# Autodesk Inventor assembly: Ensamblaje_Carcaza_sup_ch
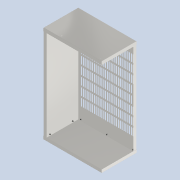
[picture p0: Inventor's stored thumbnail of the model, 180x180]
Saved by Autodesk Inventor 2021 (Build 250183000, 183)
## iProperties
Created: 2021-05-16
Part Number: Ensamblaje_Carcaza_sup_ch
Document SubType Name: Assembly
Designer: Admin
Mass: 2946.62 g
Surface Area: 11445.5 cm^2
Volume: 374.317 cm^3
Density: 7.872 g/cm^3
Author: Admin
## Documents named in this file (7)
- E:\Documentos\Documentos\Michael_Rodriguez\Universidad_Nacional\Doceaba matricula\PAI\Proyecto PAI\Proyecto_PAI_2021\01 CAD\Ensamblaje_Carcaza_sup_ch.iam
- E:\Documentos\Documentos\Michael_Rodriguez\Universidad_Nacional\Doceaba matricula\PAI\Proyecto PAI\Proyecto_PAI_2021\01 CAD\Tapa_superior_sup_ch.ipt
- E:\Documentos\Documentos\Michael_Rodriguez\Universidad_Nacional\Doceaba matricula\PAI\Proyecto PAI\Proyecto_PAI_2021\01 CAD\Tapa_superior_izq_ch.ipt
- E:\Documentos\Documentos\Michael_Rodriguez\Universidad_Nacional\Doceaba matricula\PAI\Proyecto PAI\Proyecto_PAI_2021\01 CAD\Tapa_superior_der_ch.ipt
- E:\Documentos\Documentos\Michael_Rodriguez\Universidad_Nacional\Doceaba matricula\PAI\Proyecto PAI\Proyecto_PAI_2021\01 CAD\ISO 7380-1 - M5 x 8.ipt
- E:\Documentos\Documentos\Michael_Rodriguez\Universidad_Nacional\Doceaba matricula\PAI\Proyecto PAI\Proyecto_PAI_2021\01 CAD\BS 4320 - M5 (Forma A).ipt
- E:\Documentos\Documentos\Michael_Rodriguez\Universidad_Nacional\Doceaba matricula\PAI\Proyecto PAI\Proyecto_PAI_2021\01 CAD\BS 4183 - M5(1).ipt
## Components (33 placed, 6 different names)
1. Tapa_superior_sup_ch:1 — Coincidencia:1, Coincidencia:2, Coincidencia:3, Coincidencia:4, Coincidencia:5, Coincidencia:6, De rotación:21, De rotación:22, De rotación:23, De rotación:24, De rotación:25, De rotación:26, De rotación:27, De rotación:28, De rotación:29, De rotación:30
2. Tapa_superior_izq_ch:1 — Coincidencia:4, Coincidencia:5, Coincidencia:6, De rotación:1, De rotación:2, De rotación:3, De rotación:13, De rotación:14
3. Tapa_superior_der_ch:1 — Coincidencia:1, Coincidencia:2, Coincidencia:3, De rotación:4, De rotación:5, De rotación:6, De rotación:15, De rotación:16
4. ISO 7380-1 M5 x 8:1 — De rotación:8
5. ISO 7380-1 M5 x 8:2 — De rotación:9
6. ISO 7380-1 M5 x 8:3 — De rotación:12
7. ISO 7380-1 M5 x 8:4 — De rotación:7
8. ISO 7380-1 M5 x 8:5 — De rotación:10
9. ISO 7380-1 M5 x 8:6 — De rotación:11
10. ISO 7380-1 M5 x 8:7 — De rotación:17
11. ISO 7380-1 M5 x 8:8 — De rotación:19
12. ISO 7380-1 M5 x 8:9 — De rotación:18
13. ISO 7380-1 M5 x 8:10 — De rotación:20
14. BS 4320 Forma AB M5 (Forma A):1 — De rotación:6, De rotación:12
15. BS 4320 Forma AB M5 (Forma A):2 — De rotación:5, De rotación:11
16. BS 4320 Forma AB M5 (Forma A):3 — De rotación:4, De rotación:10
17. BS 4320 Forma AB M5 (Forma A):4 — De rotación:3, De rotación:9
18. BS 4320 Forma AB M5 (Forma A):5 — De rotación:2, De rotación:8
19. BS 4320 Forma AB M5 (Forma A):6 — De rotación:1, De rotación:7
20. BS 4320 Forma AB M5 (Forma A):7 — De rotación:13, De rotación:17
21. BS 4320 Forma AB M5 (Forma A):8 — De rotación:14, De rotación:18
22. BS 4320 Forma AB M5 (Forma A):9 — De rotación:15, De rotación:20
23. BS 4320 Forma AB M5 (Forma A):10 — De rotación:16, De rotación:19
24. BS 4183 - Métrico M5:1 — De rotación:21
25. BS 4183 - Métrico M5:2 — De rotación:23
26. BS 4183 - Métrico M5:3 — De rotación:26
27. BS 4183 - Métrico M5:4 — De rotación:22
28. BS 4183 - Métrico M5:5 — De rotación:24
29. BS 4183 - Métrico M5:6 — De rotación:25
30. BS 4183 - Métrico M5:7 — De rotación:27
31. BS 4183 - Métrico M5:8 — De rotación:29
32. BS 4183 - Métrico M5:9 — De rotación:28
33. BS 4183 - Métrico M5:10 — De rotación:30
## Relationships (36: RevoluteJoint 30, Mate 6)
- Coincidencia:1 [Mate]: Tapa_superior_sup_ch:1 ↔ Tapa_superior_der_ch:1
- Coincidencia:2 [Mate]: Tapa_superior_sup_ch:1 ↔ Tapa_superior_der_ch:1
- Coincidencia:3 [Mate]: Tapa_superior_sup_ch:1 ↔ Tapa_superior_der_ch:1
- Coincidencia:4 [Mate]: Tapa_superior_sup_ch:1 ↔ Tapa_superior_izq_ch:1
- Coincidencia:5 [Mate]: Tapa_superior_sup_ch:1 ↔ Tapa_superior_izq_ch:1
- Coincidencia:6 [Mate]: Tapa_superior_sup_ch:1 ↔ Tapa_superior_izq_ch:1
- De rotación:1 [RevoluteJoint]: Tapa_superior_izq_ch:1 ↔ BS 4320 Forma AB M5 (Forma A):6
- De rotación:2 [RevoluteJoint]: Tapa_superior_izq_ch:1 ↔ BS 4320 Forma AB M5 (Forma A):5
- De rotación:3 [RevoluteJoint]: Tapa_superior_izq_ch:1 ↔ BS 4320 Forma AB M5 (Forma A):4
- De rotación:4 [RevoluteJoint]: Tapa_superior_der_ch:1 ↔ BS 4320 Forma AB M5 (Forma A):3
- De rotación:5 [RevoluteJoint]: Tapa_superior_der_ch:1 ↔ BS 4320 Forma AB M5 (Forma A):2
- De rotación:6 [RevoluteJoint]: Tapa_superior_der_ch:1 ↔ BS 4320 Forma AB M5 (Forma A):1
- De rotación:7 [RevoluteJoint]: ISO 7380-1 M5 x 8:4 ↔ BS 4320 Forma AB M5 (Forma A):6
- De rotación:8 [RevoluteJoint]: ISO 7380-1 M5 x 8:1 ↔ BS 4320 Forma AB M5 (Forma A):5
- De rotación:9 [RevoluteJoint]: ISO 7380-1 M5 x 8:2 ↔ BS 4320 Forma AB M5 (Forma A):4
- De rotación:10 [RevoluteJoint]: ISO 7380-1 M5 x 8:5 ↔ BS 4320 Forma AB M5 (Forma A):3
- De rotación:11 [RevoluteJoint]: ISO 7380-1 M5 x 8:6 ↔ BS 4320 Forma AB M5 (Forma A):2
- De rotación:12 [RevoluteJoint]: ISO 7380-1 M5 x 8:3 ↔ BS 4320 Forma AB M5 (Forma A):1
- De rotación:13 [RevoluteJoint]: Tapa_superior_izq_ch:1 ↔ BS 4320 Forma AB M5 (Forma A):7
- De rotación:14 [RevoluteJoint]: Tapa_superior_izq_ch:1 ↔ BS 4320 Forma AB M5 (Forma A):8
- De rotación:15 [RevoluteJoint]: Tapa_superior_der_ch:1 ↔ BS 4320 Forma AB M5 (Forma A):9
- De rotación:16 [RevoluteJoint]: Tapa_superior_der_ch:1 ↔ BS 4320 Forma AB M5 (Forma A):10
- De rotación:17 [RevoluteJoint]: ISO 7380-1 M5 x 8:7 ↔ BS 4320 Forma AB M5 (Forma A):7
- De rotación:18 [RevoluteJoint]: ISO 7380-1 M5 x 8:9 ↔ BS 4320 Forma AB M5 (Forma A):8
- De rotación:19 [RevoluteJoint]: ISO 7380-1 M5 x 8:8 ↔ BS 4320 Forma AB M5 (Forma A):10
- De rotación:20 [RevoluteJoint]: ISO 7380-1 M5 x 8:10 ↔ BS 4320 Forma AB M5 (Forma A):9
- De rotación:21 [RevoluteJoint]: Tapa_superior_sup_ch:1 ↔ BS 4183 - Métrico M5:1
- De rotación:22 [RevoluteJoint]: Tapa_superior_sup_ch:1 ↔ BS 4183 - Métrico M5:4
- De rotación:23 [RevoluteJoint]: Tapa_superior_sup_ch:1 ↔ BS 4183 - Métrico M5:2
- De rotación:24 [RevoluteJoint]: Tapa_superior_sup_ch:1 ↔ BS 4183 - Métrico M5:5
- De rotación:25 [RevoluteJoint]: Tapa_superior_sup_ch:1 ↔ BS 4183 - Métrico M5:6
- De rotación:26 [RevoluteJoint]: Tapa_superior_sup_ch:1 ↔ BS 4183 - Métrico M5:3
- De rotación:27 [RevoluteJoint]: Tapa_superior_sup_ch:1 ↔ BS 4183 - Métrico M5:7
- De rotación:28 [RevoluteJoint]: Tapa_superior_sup_ch:1 ↔ BS 4183 - Métrico M5:9
- De rotación:29 [RevoluteJoint]: Tapa_superior_sup_ch:1 ↔ BS 4183 - Métrico M5:8
- De rotación:30 [RevoluteJoint]: Tapa_superior_sup_ch:1 ↔ BS 4183 - Métrico M5:10
